# Autodesk Inventor assembly: Tactile_Button
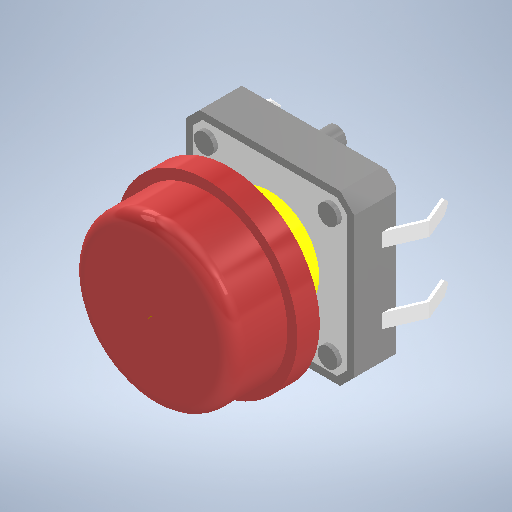
[picture p0: Inventor's stored thumbnail of the model, 512x512]
Saved by Autodesk Inventor 2025.1 (Build 291241020, 241B)
## iProperties
Created: 2024-11-21
Part Number: Tactile_Button
Document SubType Name: Assembly
Designer: leon-
Author: leon-
## Documents named in this file (3)
- C:\Users\leon-\OneDrive\Dokumente\Education\Berkeley\Embedded_Systems\Project\MagDrop4\CAD_Model\Purchase_Parts\Electronics\Tactile_Button\Tactile_Button.iam
- C:\Users\leon-\OneDrive\Dokumente\Education\Berkeley\Embedded_Systems\Project\MagDrop4\CAD_Model\Purchase_Parts\Electronics\Tactile_Button\Tactile_Button_Base.ipt
- C:\Users\leon-\OneDrive\Dokumente\Education\Berkeley\Embedded_Systems\Project\MagDrop4\CAD_Model\Purchase_Parts\Electronics\Tactile_Button\Tactile_Button_Cap.ipt
## Components (2 placed, 2 different names)
1. Tactile_Button_Base:1 — Mate:1, Mate:2
2. Tactile_Button_Cap:1 — Mate:1, Mate:2
## Relationships (2: Mate 2)
- Mate:1: Tactile_Button_Base:1 ↔ Tactile_Button_Cap:1
- Mate:2: Tactile_Button_Base:1 ↔ Tactile_Button_Cap:1
